# Autodesk Inventor assembly: Montagem1
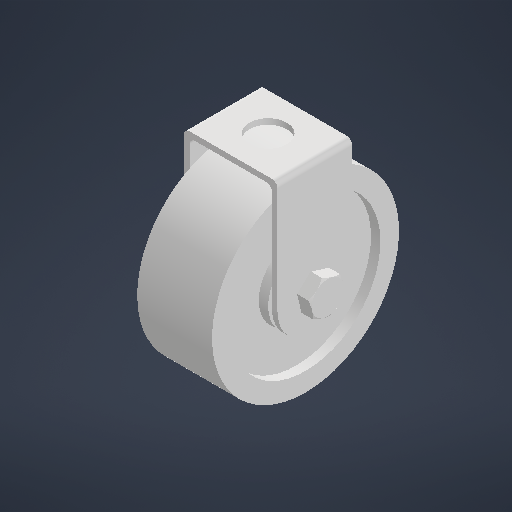
[picture p0: Inventor's stored thumbnail of the model, 512x512]
Saved by Autodesk Inventor 2027.1 (Build 311270010, 270A)
## iProperties
Created: 2026-08-27
Part Number: Montagem1
Document SubType Name: Assembly
Designer: labsfiap
Author: labsfiap
## Documents named in this file (7)
- C:\Users\labsfiap\Downloads\Montagem1.iam
- C:\Users\labsfiap\Downloads\suporte.ipt
- C:\Users\labsfiap\Downloads\rodizio.ipt
- C:\Users\labsfiap\Downloads\parafuso.ipt
- C:\Users\labsfiap\Downloads\bucha.ipt
- C:\Users\labsfiap\Downloads\arruela.ipt
- C:\Users\labsfiap\Downloads\Rosca.ipt
## Components (6 placed, 6 different names)
1. suporte:1 — Coincidente:2, Coincidente:3, Coincidente:5, Alinhado:2, Coincidente:8
2. rodizio:1 — Coincidente:1, Alinhado:1, Coincidente:3
3. parafuso:1 — Coincidente:4, Coincidente:5, Coincidente:6, Coincidente:7
4. bucha:1 — Coincidente:1, Alinhado:1, Coincidente:2, Coincidente:4
5. arruela:1 — Coincidente:6, Alinhado:2
6. Rosca:1 — Coincidente:7, Coincidente:8
## Relationships (10: Mate 8, Flush 2)
- Coincidente:1 [Mate]: rodizio:1 ↔ bucha:1
- Alinhado:1 [Flush]: rodizio:1 ↔ bucha:1
- Coincidente:2 [Mate]: suporte:1 ↔ bucha:1
- Coincidente:3 [Mate] (2 mm): suporte:1 ↔ rodizio:1
- Coincidente:4 [Mate]: parafuso:1 ↔ bucha:1
- Coincidente:5 [Mate]: suporte:1 ↔ parafuso:1
- Coincidente:6 [Mate]: parafuso:1 ↔ arruela:1
- Alinhado:2 [Flush] (-2 mm): suporte:1 ↔ arruela:1
- Coincidente:7 [Mate]: parafuso:1 ↔ Rosca:1
- Coincidente:8 [Mate] (2 mm): suporte:1 ↔ Rosca:1
